# Autodesk Inventor assembly: STL Generator
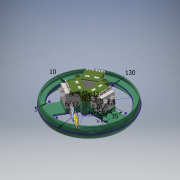
[picture p0: Inventor's stored thumbnail of the model, 180x180]
Saved by Autodesk Inventor 2018.2 (Build 222227000, 227)
## iProperties
Created: 2018-03-10
Part Number: STL Generator
Material: Generisch
Document SubType Name: Assembly
Designer: JochenAlt
Author: JochenAlt
## Documents named in this file (5)
- D:\Projects\Donna\CAD\opengl\STL Generator.iam
- D:\Projects\Donna\CAD\Donnas Head.ipt
- D:\Projects\Donna\CAD\Stewart-Base.iam
- D:\Projects\Donna\CAD\Servo-Arm-Head-20mm-Ball-Joint.iam
- D:\Projects\Donna\CAD\Stewart-Body.iam
## Components (4 placed, 4 different names)
1. Donnas Head:1 — Passend:1, Passend:2, Winkel:1
2. Stewart-Body:1 [sub-assembly] — Passend:3, Passend:4, Winkel:2
3. Servo-Arm-Head-20mm-Ball-Joint:1 [sub-assembly] — Passend:5, Passend:6, Passend:7
4. Stewart-Body-KST215MG:1 [sub-assembly] — Passend:8, Passend:9, Passend:10
## Relationships (12: Mate 10, Angle 2)
- Passend:1 [Mate]: Donnas Head:1
- Passend:2 [Mate]: Donnas Head:1
- Winkel:1 [Angle] (90 deg): Donnas Head:1
- Passend:3 [Mate]: Stewart-Body:1
- Passend:4 [Mate]: Stewart-Body:1
- Winkel:2 [Angle] (0 deg): Stewart-Body:1
- Passend:5 [Mate]: Servo-Arm-Head-20mm-Ball-Joint:1
- Passend:6 [Mate]: Servo-Arm-Head-20mm-Ball-Joint:1
- Passend:7 [Mate]: Servo-Arm-Head-20mm-Ball-Joint:1
- Passend:8 [Mate]: Stewart-Body-KST215MG:1
- Passend:9 [Mate]: Stewart-Body-KST215MG:1
- Passend:10 [Mate]: Stewart-Body-KST215MG:1
